# Autodesk Inventor assembly: Full Carousel Fixed Track Landing Gear
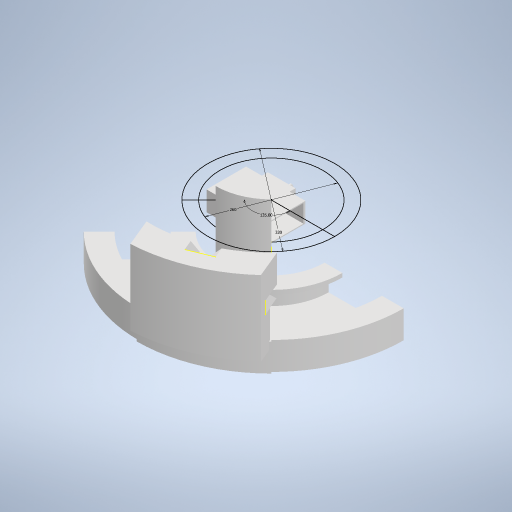
[picture p0: Inventor's stored thumbnail of the model, 512x512]
Saved by Autodesk Inventor 2023 (Build 270158000, 158)
## iProperties
Created: 2022-11-13
Part Number: Full Carousel Fixed Track Landing Gear
Document SubType Name: Assembly
Designer: mihal
Author: mihal
## Documents named in this file (4)
- C:\Users\mihal\Desktop\4th Year Project\BHSS DESIGN\Second Assembly\Full Carousel Fixed Track Landing Gear.iam
- C:\Users\mihal\Desktop\4th Year Project\BHSS DESIGN\Second Assembly\Carousel Fixed Track Landing Gear.ipt
- C:\Users\mihal\Desktop\4th Year Project\BHSS DESIGN\Second Assembly\Carousel Fixed Track.ipt
- C:\Users\mihal\Desktop\4th Year Project\BHSS DESIGN\Second Assembly\Battery Container.ipt
## Components (4 placed, 3 different names)
1. Carousel Fixed Track Landing Gear:1 — Mate:1, Mate:2, Mate:3, Mate:4, Mate:5, Mate:6
2. Carousel Fixed Track:1 — Mate:1, Mate:2, Mate:3
3. Carousel Fixed Track:2 — Mate:4, Mate:5, Mate:6
4. Battery Container:1
## Relationships (6: Mate 6)
- Mate:1: Carousel Fixed Track Landing Gear:1 ↔ Carousel Fixed Track:1
- Mate:2: Carousel Fixed Track Landing Gear:1 ↔ Carousel Fixed Track:1
- Mate:3: Carousel Fixed Track Landing Gear:1 ↔ Carousel Fixed Track:1
- Mate:4: Carousel Fixed Track Landing Gear:1 ↔ Carousel Fixed Track:2
- Mate:5: Carousel Fixed Track Landing Gear:1 ↔ Carousel Fixed Track:2
- Mate:6: Carousel Fixed Track Landing Gear:1 ↔ Carousel Fixed Track:2
